# Autodesk Inventor assembly: BoardMount
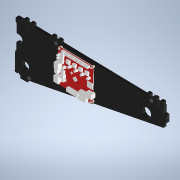
[picture p0: Inventor's stored thumbnail of the model, 180x180]
Saved by Autodesk Inventor 2020.2 (Build 242310000, 310)
## iProperties
Created: 2020-08-27
Part Number: BoardMount
Document SubType Name: Assembly
Designer: JK
Author: JK
## Documents named in this file (8)
- C:\Users\JK\Documents\Inventor\Anet Upgrade\BoardMount.iam
- C:\Users\JK\Documents\Inventor\Anet Upgrade\acrylicframepart.ipt
- C:\Users\JK\Documents\Inventor\Anet Upgrade\M5x12BoltFlatHead.ipt
- C:\Users\JK\Documents\Inventor\Anet Upgrade\T_Slot_Nut_Dropin_3030m5ipt.ipt
- C:\Users\JK\Documents\Inventor\Anet Upgrade\Anet_A8_Main_Board_shell_v1.1.ipt
- C:\Users\JK\Documents\Inventor\Anet Upgrade\Shortspacer.ipt
- C:\Users\JK\Documents\Inventor\Anet Upgrade\M3Nut.ipt
- C:\Users\JK\Documents\Inventor\Anet Upgrade\M3x20Bolt.ipt
## Components (20 placed, 7 different names)
1. acrylicframepart:1 — Mate:1, Mate:2, Mate:3, Mate:4, Angle:1, Mate:8, Angle:2, Mate:9, Mate:10, Mate:11, Mate:19, Mate:20, Mate:21, Mate:22, Mate:23, Mate:24
2. M5x12BoltFlatHead:1 — Mate:1, Flush:2, Mate:4, Mate:6
3. M5x12BoltFlatHead:2 — Mate:2, Flush:1, Flush:2, Mate:7
4. M5x12BoltFlatHead:3 — Mate:3, Flush:1, Mate:5
5. T_Slot_Nut_Dropin_3030m5ipt:1 — Mate:7, Flush:3, Angle:3
6. T_Slot_Nut_Dropin_3030m5ipt:2 — Mate:6, Flush:4, Angle:2, Angle:3
7. T_Slot_Nut_Dropin_3030m5ipt:3 — Mate:5, Flush:3, Flush:4, Angle:1, Mate:8
8. Anet_A8_Main_Board_shell_v1.1:1 — Mate:9, Mate:10, Mate:12, Mate:13, Mate:14, Mate:15, Mate:16, Mate:17, Mate:18, Mate:29
9. Shortspacer:1 — Mate:14, Mate:15, Mate:28
10. Shortspacer:2 — Mate:11, Mate:16, Mate:27
11. Shortspacer:3 — Mate:12, Mate:17, Mate:19, Mate:25
12. Shortspacer:4 — Mate:13, Mate:18, Mate:26
13. M3Nut:1 — Mate:20, Flush:5, Flush:6
14. M3Nut:2 — Mate:21, Flush:5, Mate:24
15. M3Nut:3 — Mate:22, Flush:6, Flush:7
16. M3Nut:4 — Mate:23, Flush:7
17. M3x20Bolt:1 — Mate:25, Flush:8, Flush:10, Mate:29
18. M3x20Bolt:2 — Mate:26, Flush:8, Flush:9
19. M3x20Bolt:3 — Mate:27, Flush:10
20. M3x20Bolt:4 — Mate:28, Flush:9
## Relationships (42: Mate 29, Flush 10, Angle 3)
- Mate:1: acrylicframepart:1 ↔ M5x12BoltFlatHead:1
- Mate:2: acrylicframepart:1 ↔ M5x12BoltFlatHead:2
- Mate:3: acrylicframepart:1 ↔ M5x12BoltFlatHead:3
- Flush:1: M5x12BoltFlatHead:2 ↔ M5x12BoltFlatHead:3
- Flush:2: M5x12BoltFlatHead:1 ↔ M5x12BoltFlatHead:2
- Mate:4: acrylicframepart:1 ↔ M5x12BoltFlatHead:1
- Mate:5: M5x12BoltFlatHead:3 ↔ T_Slot_Nut_Dropin_3030m5ipt:3
- Mate:6: M5x12BoltFlatHead:1 ↔ T_Slot_Nut_Dropin_3030m5ipt:2
- Mate:7: M5x12BoltFlatHead:2 ↔ T_Slot_Nut_Dropin_3030m5ipt:1
- Flush:3: T_Slot_Nut_Dropin_3030m5ipt:1 ↔ T_Slot_Nut_Dropin_3030m5ipt:3
- Flush:4: T_Slot_Nut_Dropin_3030m5ipt:2 ↔ T_Slot_Nut_Dropin_3030m5ipt:3
- Angle:1 (0 deg): acrylicframepart:1 ↔ T_Slot_Nut_Dropin_3030m5ipt:3
- Mate:8: acrylicframepart:1 ↔ T_Slot_Nut_Dropin_3030m5ipt:3
- Angle:2 (0 deg): acrylicframepart:1 ↔ T_Slot_Nut_Dropin_3030m5ipt:2
- Angle:3 (0 deg): T_Slot_Nut_Dropin_3030m5ipt:1 ↔ T_Slot_Nut_Dropin_3030m5ipt:2
- Mate:9: acrylicframepart:1 ↔ Anet_A8_Main_Board_shell_v1.1:1
- Mate:10: acrylicframepart:1 ↔ Anet_A8_Main_Board_shell_v1.1:1
- Mate:11: acrylicframepart:1 ↔ Shortspacer:2
- Mate:12: Anet_A8_Main_Board_shell_v1.1:1 ↔ Shortspacer:3
- Mate:13: Anet_A8_Main_Board_shell_v1.1:1 ↔ Shortspacer:4
- Mate:14: Anet_A8_Main_Board_shell_v1.1:1 ↔ Shortspacer:1
- Mate:15: Anet_A8_Main_Board_shell_v1.1:1 ↔ Shortspacer:1
- Mate:16: Anet_A8_Main_Board_shell_v1.1:1 ↔ Shortspacer:2
- Mate:17: Anet_A8_Main_Board_shell_v1.1:1 ↔ Shortspacer:3
- Mate:18: Anet_A8_Main_Board_shell_v1.1:1 ↔ Shortspacer:4
- Mate:19: acrylicframepart:1 ↔ Shortspacer:3
- Mate:20: acrylicframepart:1 ↔ M3Nut:1
- Mate:21: acrylicframepart:1 ↔ M3Nut:2
- Mate:22: acrylicframepart:1 ↔ M3Nut:3
- Mate:23: acrylicframepart:1 ↔ M3Nut:4
- Flush:5: M3Nut:1 ↔ M3Nut:2
- Flush:6: M3Nut:1 ↔ M3Nut:3
- Flush:7: M3Nut:3 ↔ M3Nut:4
- Mate:24: acrylicframepart:1 ↔ M3Nut:2
- Mate:25: Shortspacer:3 ↔ M3x20Bolt:1
- Mate:26: Shortspacer:4 ↔ M3x20Bolt:2
- Mate:27: Shortspacer:2 ↔ M3x20Bolt:3
- Mate:28: Shortspacer:1 ↔ M3x20Bolt:4
- Flush:8: M3x20Bolt:1 ↔ M3x20Bolt:2
- Flush:9: M3x20Bolt:2 ↔ M3x20Bolt:4
- Flush:10: M3x20Bolt:1 ↔ M3x20Bolt:3
- Mate:29: Anet_A8_Main_Board_shell_v1.1:1 ↔ M3x20Bolt:1
